# Autodesk Inventor assembly: EnclosureAssemble
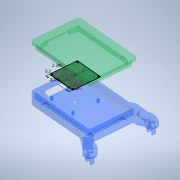
[picture p0: Inventor's stored thumbnail of the model, 180x180]
Saved by Autodesk Inventor 2020 (Build 240168000, 168)
## iProperties
Created: 2019-09-23
Part Number: EnclosureAssemble
Document SubType Name: Assembly
Designer: veloxstatera
Author: veloxstatera
## Documents named in this file (4)
- E:\smartTarget\EnclosureAssemble.iam
- E:\smartTarget\EnclosureBot.ipt
- E:\smartTarget\EnclosureTop.ipt
- E:\smartTarget\PCBboard.ipt
## Components (3 placed, 3 different names)
1. EnclosureBot:1 — Mate:3, Mate:4, Mate:5, Mate:6, Mate:7, Mate:8
2. PCBboard:1 — Mate:3, Mate:4, Mate:7, Mate:8
3. EnclosureTop:1 — Mate:5, Mate:6
## Relationships (6: Mate 6)
- Mate:3: EnclosureBot:1 ↔ PCBboard:1
- Mate:4: EnclosureBot:1 ↔ PCBboard:1
- Mate:5: EnclosureBot:1 ↔ EnclosureTop:1
- Mate:6: EnclosureBot:1 ↔ EnclosureTop:1
- Mate:7: EnclosureBot:1 ↔ PCBboard:1
- Mate:8: EnclosureBot:1 ↔ PCBboard:1
